# Autodesk Inventor assembly: balloonMount
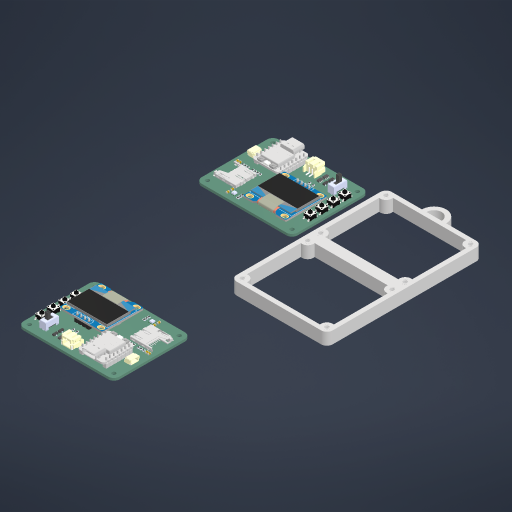
[picture p0: Inventor's stored thumbnail of the model, 512x512]
Saved by Autodesk Inventor 2024 (Build 280153000, 153)
## iProperties
Created: 2024-03-19
Part Number: balloonMount
Document SubType Name: Assembly
Designer: madis
Author: madis
## Documents named in this file (4)
- D:\Destination-SPACE-Files\development\docs\ds-weather-station-v4.5\hardware\balloonMount\balloonMount.iam
- D:\Destination-SPACE-Files\development\docs\ds-weather-station-v4.5\hardware\balloonMount\balloonMount_x2.ipt
- D:\Destination-SPACE-Files\development\docs\ds-weather-station-v4.5\hardware\balloonMount\destinationWeatherStation_v4-5\destinationWeatherStation_v4-5.iam
- D:\Destination-SPACE-Files\development\docs\ds-weather-station-v4.5\hardware\balloonMount\94180A321_Tapered Heat-Set Inserts for Plastic\94180A321_Tapered Heat-Set Inserts for Plastic.ipt
## Components (11 placed, 3 different names)
1. balloonMount_x2:1 — Mate:1, Flush:1, Mate:2, Flush:2, Mate:3, Flush:3, Mate:4, Flush:4, Mate:5, Flush:5, Mate:6, Flush:6, Mate:7, Flush:7, Mate:8, Flush:8
2. destinationWeatherStation_v4-5:1 [sub-assembly]
3. destinationWeatherStation_v4-5:2 [sub-assembly]
4. 94180A321_Tapered Heat-Set Inserts for Plastic:1 — Mate:2, Flush:2
5. 94180A321_Tapered Heat-Set Inserts for Plastic:2 — Mate:1, Flush:1
6. 94180A321_Tapered Heat-Set Inserts for Plastic:3 — Mate:5, Flush:5
7. 94180A321_Tapered Heat-Set Inserts for Plastic:4 — Mate:3, Flush:3
8. 94180A321_Tapered Heat-Set Inserts for Plastic:5 — Mate:6, Flush:6
9. 94180A321_Tapered Heat-Set Inserts for Plastic:6 — Mate:4, Flush:4
10. 94180A321_Tapered Heat-Set Inserts for Plastic:7 — Mate:8, Flush:8
11. 94180A321_Tapered Heat-Set Inserts for Plastic:8 — Mate:7, Flush:7
## Relationships (16: Mate 8, Flush 8)
- Mate:1: balloonMount_x2:1 ↔ 94180A321_Tapered Heat-Set Inserts for Plastic:2
- Flush:1: balloonMount_x2:1 ↔ 94180A321_Tapered Heat-Set Inserts for Plastic:2
- Mate:2: balloonMount_x2:1 ↔ 94180A321_Tapered Heat-Set Inserts for Plastic:1
- Flush:2: balloonMount_x2:1 ↔ 94180A321_Tapered Heat-Set Inserts for Plastic:1
- Mate:3: balloonMount_x2:1 ↔ 94180A321_Tapered Heat-Set Inserts for Plastic:4
- Flush:3: balloonMount_x2:1 ↔ 94180A321_Tapered Heat-Set Inserts for Plastic:4
- Mate:4: balloonMount_x2:1 ↔ 94180A321_Tapered Heat-Set Inserts for Plastic:6
- Flush:4: balloonMount_x2:1 ↔ 94180A321_Tapered Heat-Set Inserts for Plastic:6
- Mate:5: balloonMount_x2:1 ↔ 94180A321_Tapered Heat-Set Inserts for Plastic:3
- Flush:5: balloonMount_x2:1 ↔ 94180A321_Tapered Heat-Set Inserts for Plastic:3
- Mate:6: balloonMount_x2:1 ↔ 94180A321_Tapered Heat-Set Inserts for Plastic:5
- Flush:6: balloonMount_x2:1 ↔ 94180A321_Tapered Heat-Set Inserts for Plastic:5
- Mate:7: balloonMount_x2:1 ↔ 94180A321_Tapered Heat-Set Inserts for Plastic:8
- Flush:7: balloonMount_x2:1 ↔ 94180A321_Tapered Heat-Set Inserts for Plastic:8
- Mate:8: balloonMount_x2:1 ↔ 94180A321_Tapered Heat-Set Inserts for Plastic:7
- Flush:8: balloonMount_x2:1 ↔ 94180A321_Tapered Heat-Set Inserts for Plastic:7
